# Autodesk Inventor assembly: climber-assy
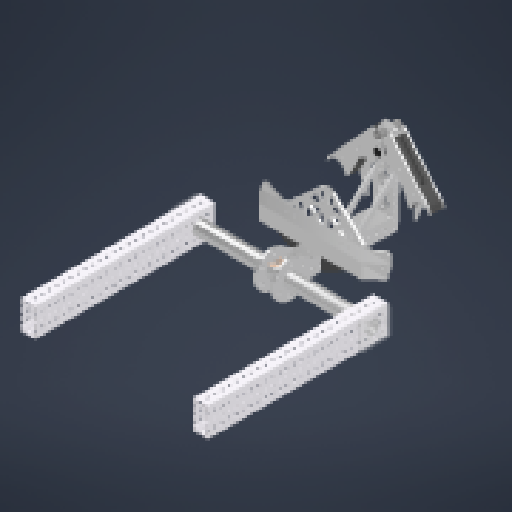
[picture p0: Inventor's stored thumbnail of the model, 512x512]
Saved by Autodesk Inventor 2025.1 (Build 291241020, 241B)
## iProperties
Category: _
Manager: _
ILogicPurgeVersion: 0.0.0.0
OnSaveVersion: 3.2.6.0
OnSaveAssembly: COREAutomationManager
Created: 2025-03-18
Part Number: climber-assy
Checked By: 00
Engr Approved By: _
User Status: Work In Process
Description: ASSY,STANDARD (mm)
Document SubType Name: Assembly
Mfg Approved By: Paul.Struhar
Designer: mathe
Mass: 1273.29 g
Surface Area: 4984.49 cm^2
Volume: 545.281 cm^3
Density: 2.3351 g/cm^3
CN_MASS: 0
CN_SERVICEABLE: _
FIRST_DESCRIPTION: _
SECOND_DESCRIPTION: _
THIRD_DESCRIPTION: _
CL_runCount: 0
ModelCat: Uncategorized
Subject: _
Author: mathe
Keywords: -
Revision Number: A
## Documents named in this file (6)
- D:\Documents\Inventor\2025-Poseidon-Mechanical\climber-assy.iam
- D:\Documents\Inventor\2025-Poseidon-Mechanical\Support,Climber,MAXTube-2x1-Holes.ipt
- D:\Documents\Inventor\2025-Poseidon-Mechanical\climber-axle.ipt
- D:\Documents\Inventor\2025-Poseidon-Mechanical\climber-axle-endcap.ipt
- D:\Documents\Inventor\2025-Poseidon-Mechanical\Assembly43.iam
- D:\Documents\Inventor\2025-Poseidon-Mechanical\grapplinghook.iam
## Components (7 placed, 5 different names)
1. Support,Climber,MAXTube-2x1-Holes:1 — Flush:1, Flush:2, Mate:1, Insert:3, Flush:4
2. Support,Climber,MAXTube-2x1-Holes:2 — Flush:1, Flush:2, Mate:1, Insert:1, Insert:2, Flush:3, Insert:4, Flush:5, Mate:2, Mate:3
3. climber-axle:1 — Insert:1
4. climber-axle-endcap:1 — Insert:2, Flush:3
5. climber-axle-endcap:2 — Insert:3, Flush:4
6. Assembly43:1 [sub-assembly]
7. grapplinghook:1 [sub-assembly] — Insert:4
## Relationships (12: Flush 5, Insert 4, Mate 3)
- Flush:1: Support,Climber,MAXTube-2x1-Holes:1 ↔ Support,Climber,MAXTube-2x1-Holes:2
- Flush:2: Support,Climber,MAXTube-2x1-Holes:1 ↔ Support,Climber,MAXTube-2x1-Holes:2
- Mate:1 (280.416 mm): Support,Climber,MAXTube-2x1-Holes:1 ↔ Support,Climber,MAXTube-2x1-Holes:2
- Insert:1: Support,Climber,MAXTube-2x1-Holes:2 ↔ climber-axle:1
- Insert:2: Support,Climber,MAXTube-2x1-Holes:2 ↔ climber-axle-endcap:1
- Flush:3: Support,Climber,MAXTube-2x1-Holes:2 ↔ climber-axle-endcap:1
- Insert:3: Support,Climber,MAXTube-2x1-Holes:1 ↔ climber-axle-endcap:2
- Flush:4: Support,Climber,MAXTube-2x1-Holes:1 ↔ climber-axle-endcap:2
- Insert:4 (120 mm): Support,Climber,MAXTube-2x1-Holes:2 ↔ grapplinghook:1
- Flush:5: Support,Climber,MAXTube-2x1-Holes:2
- Mate:2: Support,Climber,MAXTube-2x1-Holes:2
- Mate:3: Support,Climber,MAXTube-2x1-Holes:2
